# Autodesk Inventor assembly: coupler extenison arm motor+ servo mount
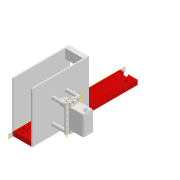
[picture p0: Inventor's stored thumbnail of the model, 180x180]
Saved by Autodesk Inventor 2020 (Build 240168000, 168)
## iProperties
Created: 2019-12-15
Part Number: coupler extenison arm motor+ servo mount
Document SubType Name: Assembly
Designer: ball
Author: ball
## Documents named in this file (4)
- C:\FTC\FTC8863CAD\2019 Robot\Delivery\extension arm\coupler extenison arm motor+ servo mount.iam
- C:\FTC\FTC8863CAD\2019 Robot\Delivery\extension arm\Coupler extension arm motor.ipt
- C:\FTC\FTC8863CAD\2019 Robot\Delivery\extension arm\whole servo mount.ipt
- C:\FTC\FTC8863CAD\2019 Robot\Delivery\extension arm\servo.iam
## Components (3 placed, 3 different names)
1. Coupler extension arm motor:1 — Flush:1, Flush:2, Flush:3, Angle:1
2. whole servo mount:1 — Flush:1, Flush:2, Flush:3, Mate:1, Mate:2
3. servo:1 [sub-assembly] — Mate:1, Mate:2, Angle:1
## Relationships (6: Flush 3, Mate 2, Angle 1)
- Flush:1: Coupler extension arm motor:1 ↔ whole servo mount:1
- Flush:2: Coupler extension arm motor:1 ↔ whole servo mount:1
- Flush:3: Coupler extension arm motor:1 ↔ whole servo mount:1
- Mate:1: whole servo mount:1 ↔ servo:1
- Mate:2: whole servo mount:1 ↔ servo:1
- Angle:1 (0 deg): Coupler extension arm motor:1 ↔ servo:1
